# Autodesk Inventor assembly: plasmaTorchAssembly
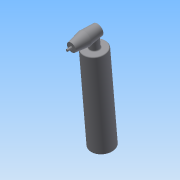
[picture p0: Inventor's stored thumbnail of the model, 180x180]
Saved by Autodesk Inventor 2015 (Build 190159000, 159)
## iProperties
Created: 2014-09-02
Part Number: plasmaTorchAssembly
Document SubType Name: Assembly
Designer: shohei
Author: shohei
## Documents named in this file (3)
- C:\Users\shohei\Documents\Inventor\PlasmaCNCrev3\Workspaces\Workspace\plasmaTorchAssembly.iam
- C:\Users\shohei\Documents\Inventor\PlasmaCNCrev3\Workspaces\Workspace\plasmatorch.ipt
- C:\Users\shohei\Documents\Inventor\PlasmaCNCrev3\Workspaces\Workspace\torchHead.ipt
## Components (2 placed, 2 different names)
1. plasmatorch:1 — Angle:1
2. torchHead:1 — Angle:1
## Relationships (1: Angle 1)
- Angle:1 (90 deg): plasmatorch:1 ↔ torchHead:1
